# Autodesk Inventor assembly: HM1
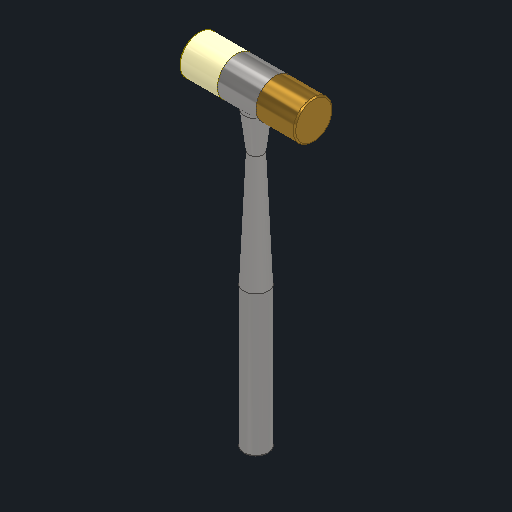
[picture p0: Inventor's stored thumbnail of the model, 512x512]
Saved by Autodesk Inventor 2024.3 (Build 283343000, 343)
## iProperties
Created: 2023-12-03
Part Number: HM1
Document SubType Name: Assembly
Designer: fablabadmin
Author: fablabadmin
## Documents named in this file (5)
- C:\Users\fablabadmin\Documents\_Benjamin_S\_3dCAD\HHVerkstad\Hammer\HM1.iam
- C:\Users\fablabadmin\Documents\_Benjamin_S\_3dCAD\HHVerkstad\Hammer\HM1-001.ipt
- C:\Users\fablabadmin\Documents\_Benjamin_S\_3dCAD\HHVerkstad\Hammer\HM1-002.ipt
- C:\Users\fablabadmin\Documents\_Benjamin_S\_3dCAD\HHVerkstad\Hammer\HM1-003A.ipt
- C:\Users\fablabadmin\Documents\_Benjamin_S\_3dCAD\HHVerkstad\Hammer\HM1-003B.ipt
## Components (4 placed, 4 different names)
1. HM1-001:1 — Mate:2, Mate:10
2. HM1-002:1 — Mate:2, Mate:3, Mate:4, Mate:5, Mate:6, Mate:7, Mate:10
3. HM1-003A:1 — Mate:4, Mate:7, Mate:8
4. HM1-003B:1 — Mate:5, Mate:6, Mate:9
## Relationships (9: Mate 9)
- Mate:2: HM1-001:1 ↔ HM1-002:1
- Mate:3: HM1-002:1
- Mate:4: HM1-002:1 ↔ HM1-003A:1
- Mate:5: HM1-002:1 ↔ HM1-003B:1
- Mate:6: HM1-002:1 ↔ HM1-003B:1
- Mate:7: HM1-002:1 ↔ HM1-003A:1
- Mate:8: HM1-003A:1
- Mate:9: HM1-003B:1
- Mate:10: HM1-001:1 ↔ HM1-002:1
